# Autodesk Inventor assembly: 3 Flex, HS
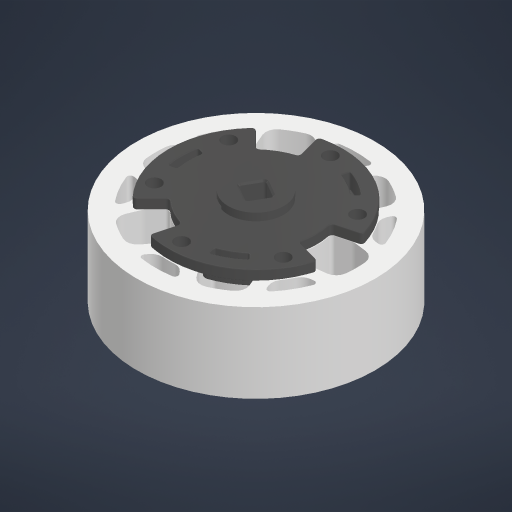
[picture p0: Inventor's stored thumbnail of the model, 512x512]
Saved by Autodesk Inventor 2023 (Build 270158000, 158)
## iProperties
Created: 2023-02-19
Part Number: 3 Flex, HS
Document SubType Name: Assembly
Designer: Windows Macbook
Author: Windows Macbook
## Documents named in this file (5)
- C:\Users\Windows Macbook\Desktop\Inventor\Motion\Wheels\Flex Wheels\3 Flex, HS.iam
- C:\Users\Windows Macbook\Desktop\Inventor\Motion\Wheels\Flex Wheels\3.000 Flex Wheel\3.000 30A 1.000.ipt
- C:\Users\Windows Macbook\Desktop\Inventor\Motion\Wheels\Flex Wheels\3.000 Flex Wheel.ipt
- C:\Users\Windows Macbook\Desktop\Inventor\Motion\Wheels\Flex Wheels\VersaHub.ipt
- C:\Users\Windows Macbook\Desktop\Inventor\Motion\Wheels\Flex Wheels\VersaHex Adapters .250.ipt
## Components (5 placed, 3 different names)
1. 3.000 30A 1.000:1 — Insert:3, Insert:4, Insert:5, Insert:6
2. VersaHub:1 — Insert:3, Insert:4
3. VersaHex Adapters .250:1
4. VersaHub:2 — Insert:5, Insert:6, Mate:2
5. VersaHex Adapters .250:2 — Mate:2
## Relationships (8: Insert 6, Mate 2)
- [Insert]: VersaHub:1 ↔ VersaHex Adapters .250:1
- [Mate]: VersaHub:1 ↔ VersaHex Adapters .250:1
- [Insert]: VersaHub:2 ↔ VersaHex Adapters .250:2
- Insert:3: 3.000 30A 1.000:1 ↔ VersaHub:1
- Insert:4: 3.000 30A 1.000:1 ↔ VersaHub:1
- Insert:5: 3.000 30A 1.000:1 ↔ VersaHub:2
- Insert:6: 3.000 30A 1.000:1 ↔ VersaHub:2
- Mate:2: VersaHub:2 ↔ VersaHex Adapters .250:2
## Named parameters: d5_d3 = 0 mm
